# Autodesk Inventor assembly: Sport57 w Redline Motor 100_1
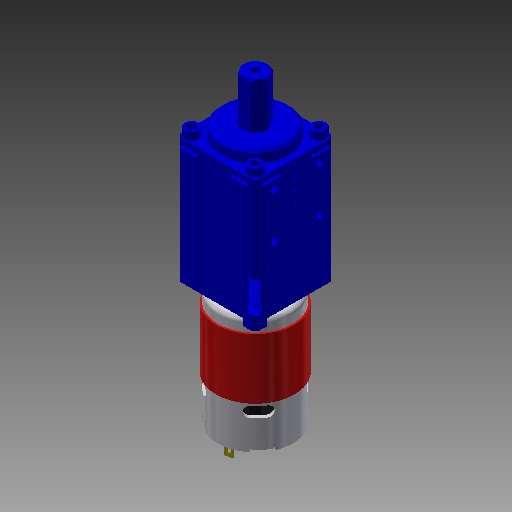
[picture p0: Inventor's stored thumbnail of the model, 512x512]
Saved by Autodesk Inventor 2018 (Build 220112000, 112)
## iProperties
Created: 2018-01-29
Part Number: Sport57 w Redline Motor 100_1
Document SubType Name: Assembly
Designer: Apple
Author: Apple
## Documents named in this file (3)
- C:\Users\Apple\Documents\Inventor\2018 PowerUp\AndyMark\Sport57 w Redline Motor 100_1.iam
- C:\Users\Apple\Documents\Inventor\2018 PowerUp\AndyMark\am-3758+-+100_1+-+57+Sport.ipt
- C:\Users\Apple\Documents\Inventor\2018 PowerUp\AndyMark\am-3775+RedLine+Motor.ipt
## Components (2 placed, 2 different names)
1. am-3758+-+100_1+-+57+Sport:1 — Mate:1, Mate:2
2. am-3775+RedLine+Motor:1 — Mate:1, Mate:2
## Relationships (2: Mate 2)
- Mate:1: am-3758+-+100_1+-+57+Sport:1 ↔ am-3775+RedLine+Motor:1
- Mate:2: am-3758+-+100_1+-+57+Sport:1 ↔ am-3775+RedLine+Motor:1
